# Autodesk Inventor assembly: Servo Asem
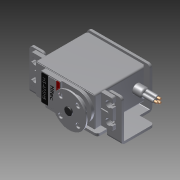
[picture p0: Inventor's stored thumbnail of the model, 180x180]
Saved by Autodesk Inventor 2011 (Build 150239000, 239)
## iProperties
Created: 2010-11-01
Part Number: Servo Asem
Document SubType Name: Assembly
Designer: AndrewRemmers
Author: AndrewRemmers
## Documents named in this file (3)
- C:\Users\AndrewRemmers\Documents\Inventor\FTC 2010 GET OVER IT\FTC CAD Database\FTC CAD Files\Servos\Servo Asem.iam
- C:\Users\AndrewRemmers\Documents\Inventor\FTC 2010 GET OVER IT\Imported Components\Single Servo Mount\Part26.ipt
- C:\Users\AndrewRemmers\Documents\Inventor\FTC 2010 GET OVER IT\Imported Components\180 Degree Servo\Assembly3.iam
## Components (2 placed, 2 different names)
1. Part26:1 — Mate:1, Flush:1, Flush:2
2. Assembly3:1 [sub-assembly] — Mate:1, Flush:1, Flush:2
## Relationships (3: Flush 2, Mate 1)
- Mate:1: Part26:1 ↔ Assembly3:1
- Flush:1 (0.508 mm): Part26:1 ↔ Assembly3:1
- Flush:2 (3.556 mm): Part26:1 ↔ Assembly3:1
